# Autodesk Inventor assembly: sindouki_assem v1
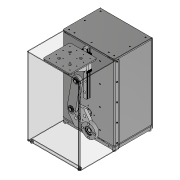
[picture p0: Inventor's stored thumbnail of the model, 180x180]
Saved by Autodesk Inventor 2020 (Build 240168000, 168)
## iProperties
Created: 2021-08-17
Part Number: sindouki_assem v1
Document SubType Name: Assembly
Designer: ken113
Sending System: Autodesk Translation Framework v10.9.0.1377
Preprocessor: ST-DEVELOPER v18.1
Title: D:/Downloads/sindouki_assem v1.step
## Documents named in this file (23)
- C:\Users\lvglv\Documents\GitHub\Vibration_Generator\Parts\Sample\sindouki_assem v1.iam
- C:\Users\lvglv\Documents\GitHub\Vibration_Generator\Parts\Sample\A1816_F v1.ipt
- C:\Users\lvglv\Documents\GitHub\Vibration_Generator\Parts\Sample\SOL5M8F v1.ipt
- C:\Users\lvglv\Documents\GitHub\Vibration_Generator\Parts\Sample\part1 v1.ipt
- C:\Users\lvglv\Documents\GitHub\Vibration_Generator\Parts\Sample\part2 v1.ipt
- C:\Users\lvglv\Documents\GitHub\Vibration_Generator\Parts\Sample\MCOC30-12-14 v1.iam
- C:\Users\lvglv\Documents\GitHub\Vibration_Generator\Parts\Sample\BGRAB6001ZZ v1.iam
- C:\Users\lvglv\Documents\GitHub\Vibration_Generator\Parts\Sample\part4 v1.ipt
- C:\Users\lvglv\Documents\GitHub\Vibration_Generator\Parts\Sample\part5 v1.ipt
- C:\Users\lvglv\Documents\GitHub\Vibration_Generator\Parts\Sample\100_100 v1.ipt
- C:\Users\lvglv\Documents\GitHub\Vibration_Generator\Parts\Sample\main_cover v1.ipt
- C:\Users\lvglv\Documents\GitHub\Vibration_Generator\Parts\Sample\HFS6-3030-272 v1.ipt
- C:\Users\lvglv\Documents\GitHub\Vibration_Generator\Parts\Sample\SFL6800ZZ v1.ipt
- C:\Users\lvglv\Documents\GitHub\Vibration_Generator\Parts\Sample\PACK10-CIMRS12-15-0.5 v1.ipt
- C:\Users\lvglv\Documents\GitHub\Vibration_Generator\Parts\Sample\SSTHR12-MB v1.iam
- C:\Users\lvglv\Documents\GitHub\Vibration_Generator\Parts\Meviy\Flange.ipt
- C:\Users\lvglv\Documents\GitHub\Vibration_Generator\Parts\Meviy\Plate_Angle.ipt
- C:\Users\lvglv\Documents\GitHub\Vibration_Generator\Parts\MISUMI\C-SXR24-160_Autodesk_Inventor_2020_20210817\AIS2020\C-SXR24-160.iam
- C:\Users\lvglv\Documents\GitHub\Vibration_Generator\Parts\MISUMI\C-30-RK-10-EP-UL-BLACK_STEP\C-30-RK-10-EP-UL-BLACK.ipt
- C:\Users\lvglv\Documents\GitHub\Vibration_Generator\Parts\Meviy\Cover_A.ipt
- C:\Users\lvglv\Documents\GitHub\Vibration_Generator\Parts\MISUMI\SSFRBF-D10-L22.5-M5-U3_Autodesk_Inventor_2020_20210817\SSFRBF-D10-L22_5-M5-U3.ipt
- C:\Users\lvglv\Documents\GitHub\Vibration_Generator\Parts\MISUMI\PSSFG12-63-RC22_Autodesk_Inventor_2020_20210817\PSSFG12-63-RC22.ipt
- C:\Users\lvglv\Documents\GitHub\Vibration_Generator\Parts\MISUMI\STWN10_Autodesk_Inventor_2020_20210817\STWN10.ipt
## Components (37 placed, 22 different names)
1. A1816_F v1:1 — 挿入:42
2. SOL5M8F v1:1 — 挿入:15, 挿入:16
3. part1 v1:2 — メイト:14, 角度:2, 挿入:28, メイト:16, 挿入:29, 挿入:30, メイト:18, 挿入:37, メイト:19, メイト:20, 挿入:44
4. part2 v1:1 — 挿入:13, 挿入:14, 角度:1, 挿入:15, 挿入:16, 挿入:29, 挿入:30, 挿入:31, 挿入:32, 挿入:33, 挿入:34, 挿入:35, 挿入:36, フラッシュ:3
5. part4 v1:1 — 挿入:21, メイト:10, フラッシュ:2, 挿入:25, 挿入:26, 挿入:27, メイト:15, 挿入:41
6. part5 v1:1 — 挿入:1, 挿入:2, 挿入:5, 挿入:6
7. 100*100 v1:1 — メイト:13, 挿入:47
8. main_cover v1:1 — メイト:18, 挿入:37
9. HFS6-3030-272 v1:1 — 挿入:13, フラッシュ:1
10. HFS6-3030-272 v1:2 — 挿入:14, 角度:1, フラッシュ:1
11. SFL6800ZZ v1:2 — 挿入:2, 挿入:3
12. SFL6800ZZ v1:4 — 挿入:6, 挿入:8
13. SFL6800ZZ v1:6 — 挿入:5
14. SFL6800ZZ v1:7 — 挿入:1, メイト:6
15. PACK10-CIMRS12-15-0.5 v1:1 — 挿入:8, 挿入:21
16. PACK10-CIMRS12-15-0.5 v1:2 — 挿入:3, メイト:5
17. SSTHR12-MB v1:1 [sub-assembly] — 挿入:20, メイト:4
18. Flange:1 — 挿入:20, メイト:4, メイト:5, メイト:6, 挿入:43
19. Plate_Angle:1 — メイト:10, フラッシュ:2, メイト:13, 挿入:25, 挿入:26, 挿入:47
20. C-SXR24-160:1 [sub-assembly] — メイト:14, 挿入:27, メイト:15, 角度:2, 挿入:28, メイト:16
21. C-30-RK-10-EP-UL-BLACK:1 — 挿入:33
22. C-30-RK-10-EP-UL-BLACK:2 — 挿入:34
23. C-30-RK-10-EP-UL-BLACK:3 — 挿入:35
24. C-30-RK-10-EP-UL-BLACK:4 — 挿入:31
25. C-30-RK-10-EP-UL-BLACK:5 — 挿入:32
26. C-30-RK-10-EP-UL-BLACK:6 — 挿入:36
27. Cover_A:1 — メイト:19, フラッシュ:3, メイト:20, 挿入:38, 挿入:39
28. C-30-RK-10-EP-UL-BLACK:7 — 挿入:38
29. C-30-RK-10-EP-UL-BLACK:8 — 挿入:39
30. SSFRBF-D10-L22_5-M5-U3:1 — 挿入:45
31. SSFRBF-D10-L22_5-M5-U3:2 — 挿入:41, 挿入:46
32. MCOC30-12-14 v1:2 [sub-assembly] — 挿入:42, メイト:22
33. PSSFG12-63-RC22:2 — 挿入:43, メイト:21, メイト:22
34. BGRAB6001ZZ v1:2 [sub-assembly]
35. BGRAB6001ZZ v1:3 [sub-assembly] — 挿入:44, メイト:21
36. STWN10:1 — 挿入:45
37. STWN10:2 — 挿入:46
## Relationships (53: Insert 35, Mate 13, Flush 3, Angle 2)
- 挿入:1 [Insert]: part5 v1:1 ↔ SFL6800ZZ v1:7
- 挿入:2 [Insert]: part5 v1:1 ↔ SFL6800ZZ v1:2
- 挿入:3 [Insert]: SFL6800ZZ v1:2 ↔ PACK10-CIMRS12-15-0.5 v1:2
- 挿入:5 [Insert]: part5 v1:1 ↔ SFL6800ZZ v1:6
- 挿入:6 [Insert]: part5 v1:1 ↔ SFL6800ZZ v1:4
- 挿入:8 [Insert]: SFL6800ZZ v1:4 ↔ PACK10-CIMRS12-15-0.5 v1:1
- 挿入:13 [Insert]: part2 v1:1 ↔ HFS6-3030-272 v1:1
- 挿入:14 [Insert]: part2 v1:1 ↔ HFS6-3030-272 v1:2
- 角度:1 [Angle] (0 deg): part2 v1:1 ↔ HFS6-3030-272 v1:2
- フラッシュ:1 [Flush]: HFS6-3030-272 v1:1 ↔ HFS6-3030-272 v1:2
- 挿入:15 [Insert]: SOL5M8F v1:1 ↔ part2 v1:1
- 挿入:16 [Insert]: SOL5M8F v1:1 ↔ part2 v1:1
- 挿入:20 [Insert]: SSTHR12-MB v1:1 ↔ Flange:1
- メイト:4 [Mate]: SSTHR12-MB v1:1 ↔ Flange:1
- メイト:5 [Mate]: PACK10-CIMRS12-15-0.5 v1:2 ↔ Flange:1
- メイト:6 [Mate]: SFL6800ZZ v1:7 ↔ Flange:1
- 挿入:21 [Insert]: part4 v1:1 ↔ PACK10-CIMRS12-15-0.5 v1:1
- メイト:10 [Mate]: part4 v1:1 ↔ Plate_Angle:1
- フラッシュ:2 [Flush]: part4 v1:1 ↔ Plate_Angle:1
- メイト:13 [Mate]: 100*100 v1:1 ↔ Plate_Angle:1
- 挿入:25 [Insert]: part4 v1:1 ↔ Plate_Angle:1
- 挿入:26 [Insert]: part4 v1:1 ↔ Plate_Angle:1
- メイト:14 [Mate]: part1 v1:2 ↔ C-SXR24-160:1
- 挿入:27 [Insert]: part4 v1:1 ↔ C-SXR24-160:1
- メイト:15 [Mate]: part4 v1:1 ↔ C-SXR24-160:1
- 角度:2 [Angle] (0 deg): part1 v1:2 ↔ C-SXR24-160:1
- 挿入:28 [Insert]: part1 v1:2 ↔ C-SXR24-160:1
- メイト:16 [Mate]: part1 v1:2 ↔ C-SXR24-160:1
- 挿入:29 [Insert]: part1 v1:2 ↔ part2 v1:1
- 挿入:30 [Insert]: part1 v1:2 ↔ part2 v1:1
- 挿入:31 [Insert]: part2 v1:1 ↔ C-30-RK-10-EP-UL-BLACK:4
- 挿入:32 [Insert]: part2 v1:1 ↔ C-30-RK-10-EP-UL-BLACK:5
- 挿入:33 [Insert]: part2 v1:1 ↔ C-30-RK-10-EP-UL-BLACK:1
- 挿入:34 [Insert]: part2 v1:1 ↔ C-30-RK-10-EP-UL-BLACK:2
- 挿入:35 [Insert]: part2 v1:1 ↔ C-30-RK-10-EP-UL-BLACK:3
- 挿入:36 [Insert]: part2 v1:1 ↔ C-30-RK-10-EP-UL-BLACK:6
- メイト:18 [Mate]: part1 v1:2 ↔ main_cover v1:1
- 挿入:37 [Insert]: part1 v1:2 ↔ main_cover v1:1
- メイト:19 [Mate]: part1 v1:2 ↔ Cover_A:1
- フラッシュ:3 [Flush]: part2 v1:1 ↔ Cover_A:1
- メイト:20 [Mate] (-12 mm): part1 v1:2 ↔ Cover_A:1
- 挿入:38 [Insert]: Cover_A:1 ↔ C-30-RK-10-EP-UL-BLACK:7
- 挿入:39 [Insert]: Cover_A:1 ↔ C-30-RK-10-EP-UL-BLACK:8
- [Insert]: Flange:1 ↔ SSFRBF-D10-L22_5-M5-U3:1
- 挿入:41 [Insert]: part4 v1:1 ↔ SSFRBF-D10-L22_5-M5-U3:2
- 挿入:42 [Insert]: A1816_F v1:1 ↔ MCOC30-12-14 v1:2
- 挿入:43 [Insert]: Flange:1 ↔ PSSFG12-63-RC22:2
- 挿入:44 [Insert]: part1 v1:2 ↔ BGRAB6001ZZ v1:3
- メイト:21 [Mate]: PSSFG12-63-RC22:2 ↔ BGRAB6001ZZ v1:3
- メイト:22 [Mate]: MCOC30-12-14 v1:2 ↔ PSSFG12-63-RC22:2
- 挿入:45 [Insert]: SSFRBF-D10-L22_5-M5-U3:1 ↔ STWN10:1
- 挿入:46 [Insert]: SSFRBF-D10-L22_5-M5-U3:2 ↔ STWN10:2
- 挿入:47 [Insert]: 100*100 v1:1 ↔ Plate_Angle:1
